# Autodesk Inventor assembly: Vacubot v1
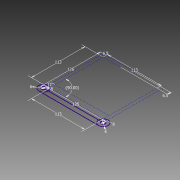
[picture p0: Inventor's stored thumbnail of the model, 180x180]
Saved by Autodesk Inventor 2014 SP1 (Build 180222100, 222)
## iProperties
Created: 2013-12-26
Part Number: Vacubot v1
Document SubType Name: Assembly
Designer: tom
Author: tom
## Documents named in this file (3)
- C:\Users\tom\Documents\GitHub\Vacubot\Inventor\Vacubot v1.iam
- C:\Users\tom\Documents\GitHub\Vacubot\Inventor\Base.ipt
- C:\Users\tom\Documents\GitHub\Vacubot\Inventor\Lower Rack Mount.ipt
## Components (2 placed, 2 different names)
1. Base:1
2. Lower Rack Mount:1 — Flush:1
## Relationships (1: Flush 1)
- Flush:1: Lower Rack Mount:1
